# Autodesk Inventor assembly: 1.7assem
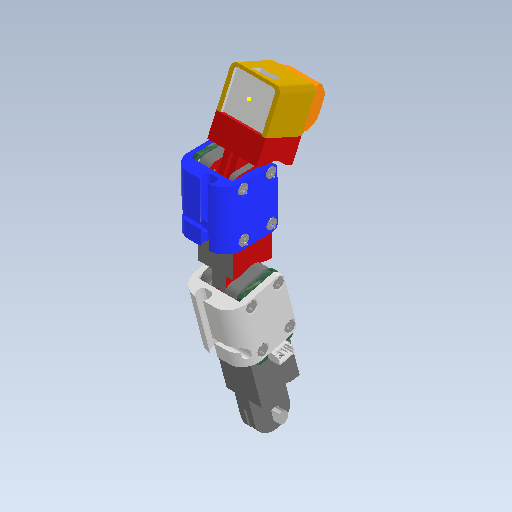
[picture p0: Inventor's stored thumbnail of the model, 512x512]
Saved by Autodesk Inventor 2020 (Build 240168000, 168)
## iProperties
Created: 2020-01-20
Part Number: 1.7assem
Document SubType Name: Assembly
Designer: sami_
Author: sami_
## Documents named in this file (4)
- C:\Users\sami_\Documents\V1.6\Workgroups\NotInProject\INDEX\finger INDEX.iam
- C:\Users\sami_\Documents\V1.6\Workgroups\NotInProject\INDEX\Fingertip assembly final.iam
- C:\Users\sami_\Documents\V1.6\IndexL1.iam
- C:\Users\sami_\Documents\V1.6\IndexL2.iam
## Components (3 placed, 3 different names)
1. Fingertip assembly final:1 [sub-assembly] — Rotational:27
2. IndexL1:1 [sub-assembly]
3. IndexL2:1 [sub-assembly] — Rotational:27
## Relationships (5: Mate 3, RevoluteJoint 2)
- [RevoluteJoint]: IndexL1:1 ↔ IndexL2:1
- [Mate]: IndexL2:1
- [Mate]: IndexL2:1
- Rotational:27 [RevoluteJoint] (0.8 mm): Fingertip assembly final:1 ↔ IndexL2:1
- [Mate]: IndexL1:1 ↔ IndexL2:1
